# Autodesk Inventor assembly: UltrasonicAssembly
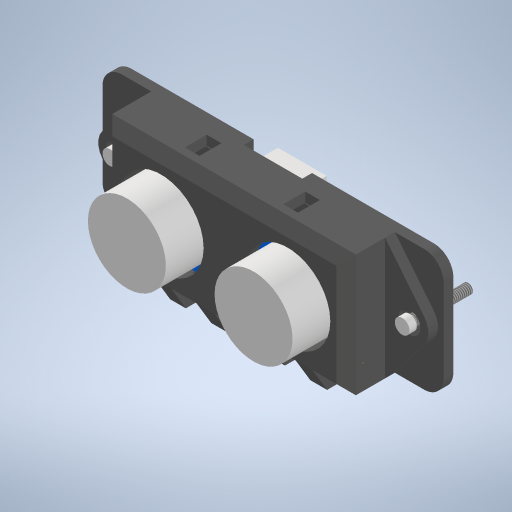
[picture p0: Inventor's stored thumbnail of the model, 512x512]
Saved by Autodesk Inventor 2024.2 (Build 282272000, 272)
## iProperties
Created: 2024-05-04
Part Number: UltrasonicAssembly
Document SubType Name: Assembly
Designer: ringl
Author: ringl
## Documents named in this file (6)
- C:\Users\ringl\OneDrive\Uni_PC_backup\Y4S2\EE579\Assignment\EE579-Skittles\CAD\Assembly\Main\UltrasonicAssembly.iam
- C:\Users\ringl\OneDrive\Uni_PC_backup\Y4S2\EE579\Assignment\EE579-Skittles\CAD\UltrasonicSensorMount02.ipt
- C:\Users\ringl\OneDrive\Uni_PC_backup\Y4S2\EE579\Assignment\EE579-Skittles\CAD\Components\UltrasonicSensor.ipt
- C:\Users\ringl\OneDrive\Uni_PC_backup\Y4S2\EE579\Assignment\EE579-Skittles\CAD\UltrasonicSensorMount_backplate03.ipt
- C:\Users\ringl\OneDrive\Uni_PC_backup\Y4S2\EE579\Assignment\EE579-Skittles\CAD\Components\M2x12.ipt
- C:\Users\ringl\OneDrive\Uni_PC_backup\Y4S2\EE579\Assignment\EE579-Skittles\CAD\Components\M2Nut.ipt
## Components (7 placed, 5 different names)
1. UltrasonicSensorMount02:1 — Mate:3, Mate:4, Mate:5, Mate:6, Mate:7, Mate:8, Mate:10, Mate:11, Mate:12
2. UltrasonicSensorMount_backplate03:1 — Mate:3, Mate:4, Mate:5, Mate:9, Mate:14, Mate:15
3. UltrasonicSensor:1 — Mate:6, Mate:7, Mate:8
4. M2x12:1 — Mate:9, Mate:12, Mate:16
5. M2x12:2 — Mate:10, Mate:11, Mate:13
6. M2Nut:1 — Mate:13, Mate:14
7. M2Nut:2 — Mate:15, Mate:16
## Relationships (14: Mate 14)
- Mate:3: UltrasonicSensorMount02:1 ↔ UltrasonicSensorMount_backplate03:1
- Mate:4: UltrasonicSensorMount02:1 ↔ UltrasonicSensorMount_backplate03:1
- Mate:5: UltrasonicSensorMount02:1 ↔ UltrasonicSensorMount_backplate03:1
- Mate:6: UltrasonicSensorMount02:1 ↔ UltrasonicSensor:1
- Mate:7: UltrasonicSensorMount02:1 ↔ UltrasonicSensor:1
- Mate:8: UltrasonicSensorMount02:1 ↔ UltrasonicSensor:1
- Mate:9: UltrasonicSensorMount_backplate03:1 ↔ M2x12:1
- Mate:10: UltrasonicSensorMount02:1 ↔ M2x12:2
- Mate:11: UltrasonicSensorMount02:1 ↔ M2x12:2
- Mate:12: UltrasonicSensorMount02:1 ↔ M2x12:1
- Mate:13: M2x12:2 ↔ M2Nut:1
- Mate:14: UltrasonicSensorMount_backplate03:1 ↔ M2Nut:1
- Mate:15: UltrasonicSensorMount_backplate03:1 ↔ M2Nut:2
- Mate:16: M2x12:1 ↔ M2Nut:2
